# Autodesk Inventor assembly: FullAsm
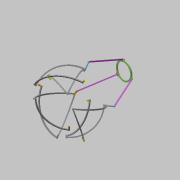
[picture p0: Inventor's stored thumbnail of the model, 180x180]
Saved by Autodesk Inventor 2015 (Build 190159000, 159)
## iProperties
Created: 2016-06-12
Part Number: FullAsm
Document SubType Name: Assembly
Designer: kumagai
Author: kumagai
## Documents named in this file (10)
- C:\home\kumagai\Develop\CAD\Para_3USR\FullAsm.iam
- C:\home\kumagai\Develop\CAD\Para_3USR\BaseAxes.ipt
- C:\home\kumagai\Develop\CAD\Para_3USR\ArcFrame\ArcFrameRd.ipt
- C:\home\kumagai\Develop\CAD\Para_3USR\ArcFrame.ipt
- C:\home\kumagai\Develop\CAD\Para_3USR\ArcFrame\ArcFrameRa.ipt
- C:\home\kumagai\Develop\CAD\Para_3USR\ArcFrame\ArcFrameRc.ipt
- C:\home\kumagai\Develop\CAD\Para_3USR\ArcFrame\ArcFrameRb.ipt
- C:\home\kumagai\Develop\CAD\Para_3USR\LinkPin.ipt
- C:\home\kumagai\Develop\CAD\Para_3USR\LinkRod.ipt
- C:\home\kumagai\Develop\CAD\Para_3USR\EndEffector.ipt
## Components (20 placed, 8 different names)
1. BaseAxes:1 — 回転:1, 回転:2, 回転:3, 回転:4, 回転:5, 回転:6
2. ArcFrameRd:1 — 回転:1, 回転:7
3. ArcFrameRd:2 — 回転:2, 回転:8
4. ArcFrameRd:3 — 回転:3, 回転:9
5. ArcFrameRa:4 — 回転:4, 回転:10
6. ArcFrameRa:5 — 回転:5, 回転:11
7. ArcFrameRa:6 — 回転:6, 回転:12
8. ArcFrameRc:7 — 回転:7, 回転:13, 回転:16
9. ArcFrameRc:8 — 回転:8, 回転:14, 回転:17
10. ArcFrameRc:9 — 回転:9, 回転:15, 回転:18
11. ArcFrameRb:10 — 回転:10, 回転:13
12. ArcFrameRb:11 — 回転:11, 回転:14
13. ArcFrameRb:12 — 回転:12, 回転:15
14. LinkPin:1 — 回転:16, ボール:1
15. LinkPin:2 — 回転:17, ボール:2
16. LinkPin:3 — 回転:18, ボール:3
17. LinkRod:1 — ボール:1, 回転:19
18. LinkRod:2 — ボール:2, 回転:20
19. LinkRod:3 — ボール:3, 回転:21
20. EndEffector:1 — 回転:19, 回転:20, 回転:21
## Relationships (24: RevoluteJoint 21, BallJoint 3)
- 回転:1 [RevoluteJoint]: BaseAxes:1 ↔ ArcFrameRd:1
- 回転:2 [RevoluteJoint]: BaseAxes:1 ↔ ArcFrameRd:2
- 回転:3 [RevoluteJoint]: BaseAxes:1 ↔ ArcFrameRd:3
- 回転:4 [RevoluteJoint]: BaseAxes:1 ↔ ArcFrameRa:4
- 回転:5 [RevoluteJoint]: BaseAxes:1 ↔ ArcFrameRa:5
- 回転:6 [RevoluteJoint]: BaseAxes:1 ↔ ArcFrameRa:6
- 回転:7 [RevoluteJoint]: ArcFrameRd:1 ↔ ArcFrameRc:7
- 回転:8 [RevoluteJoint]: ArcFrameRd:2 ↔ ArcFrameRc:8
- 回転:9 [RevoluteJoint]: ArcFrameRd:3 ↔ ArcFrameRc:9
- 回転:10 [RevoluteJoint]: ArcFrameRa:4 ↔ ArcFrameRb:10
- 回転:11 [RevoluteJoint]: ArcFrameRa:5 ↔ ArcFrameRb:11
- 回転:12 [RevoluteJoint]: ArcFrameRa:6 ↔ ArcFrameRb:12
- 回転:13 [RevoluteJoint]: ArcFrameRc:7 ↔ ArcFrameRb:10
- 回転:14 [RevoluteJoint]: ArcFrameRc:8 ↔ ArcFrameRb:11
- 回転:15 [RevoluteJoint]: ArcFrameRc:9 ↔ ArcFrameRb:12
- 回転:16 [RevoluteJoint]: ArcFrameRc:7 ↔ LinkPin:1
- 回転:17 [RevoluteJoint]: ArcFrameRc:8 ↔ LinkPin:2
- 回転:18 [RevoluteJoint]: ArcFrameRc:9 ↔ LinkPin:3
- ボール:1 [BallJoint]: LinkPin:1 ↔ LinkRod:1
- ボール:2 [BallJoint]: LinkPin:2 ↔ LinkRod:2
- ボール:3 [BallJoint]: LinkPin:3 ↔ LinkRod:3
- 回転:19 [RevoluteJoint]: LinkRod:1 ↔ EndEffector:1
- 回転:20 [RevoluteJoint]: LinkRod:2 ↔ EndEffector:1
- 回転:21 [RevoluteJoint]: LinkRod:3 ↔ EndEffector:1
